# Autodesk Inventor assembly: belt_liner-2-1
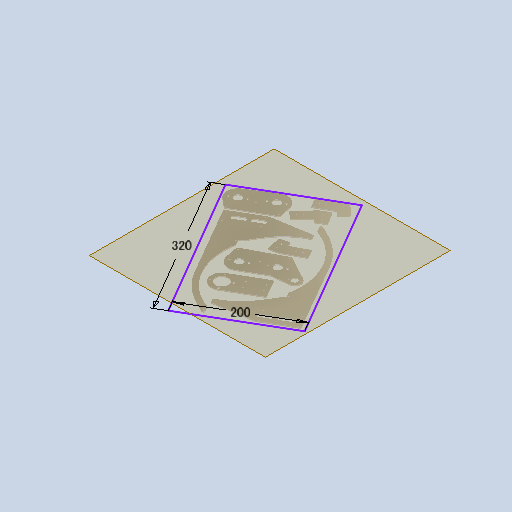
[picture p0: Inventor's stored thumbnail of the model, 512x512]
Saved by Autodesk Inventor 2025.2 (Build 292293000, 293)
## iProperties
Created: 2025-01-15
Part Number: belt_liner-2-1
Document SubType Name: Assembly
Designer: haruy
Author: haruy
## Documents named in this file (7)
- C:\Users\haruy\Documents\ロボコン\NHK2025\cad\cnc\belt_liner-2-1.iam
- C:\Users\haruy\Documents\ロボコン\NHK2025\cad\nagahisa\belt_liner\belt_liner_v2_Plate_6.ipt
- C:\Users\haruy\Documents\ロボコン\NHK2025\cad\nagahisa\belt_liner\belt_liner_v2_Plate_15.ipt
- C:\Users\haruy\Documents\ロボコン\NHK2025\cad\nagahisa\belt_liner\belt_liner_v2_Plate_17.ipt
- C:\Users\haruy\Documents\ロボコン\NHK2025\cad\nagahisa\belt_liner\belt_liner_v2_Plate_16.ipt
- C:\Users\haruy\Documents\ロボコン\NHK2025\cad\nagahisa\dribl\dribl-v1-Plate-10.ipt
- C:\Users\haruy\Documents\ロボコン\NHK2025\cad\nagahisa\dribl\dribl-v1-Plate-11.ipt
## Components (8 placed, 6 different names)
1. belt_liner_v2_Plate_6:1 — フラッシュ:1, 角度:1, 角度:2, 角度:3
2. belt_liner_v2_Plate_6:2 — フラッシュ:2, 角度:1, メイト:1
3. belt_liner_v2_Plate_15:1 — フラッシュ:3, 角度:2
4. belt_liner_v2_Plate_17:1 — フラッシュ:4, メイト:2
5. belt_liner_v2_Plate_16:1 — フラッシュ:5, メイト:1
6. dribl-v1-Plate-10:1 — フラッシュ:6, メイト:2
7. dribl-v1-Plate-10:2 — フラッシュ:7, 角度:3, メイト:3
8. dribl-v1-Plate-11:1 — フラッシュ:8, メイト:3
## Relationships (14: Flush 8, Angle 3, Mate 3)
- フラッシュ:1 [Flush]: belt_liner_v2_Plate_6:1
- フラッシュ:2 [Flush]: belt_liner_v2_Plate_6:2
- 角度:1 [Angle] (180 deg): belt_liner_v2_Plate_6:1 ↔ belt_liner_v2_Plate_6:2
- フラッシュ:3 [Flush]: belt_liner_v2_Plate_15:1
- 角度:2 [Angle] (0 deg): belt_liner_v2_Plate_6:1 ↔ belt_liner_v2_Plate_15:1
- フラッシュ:4 [Flush]: belt_liner_v2_Plate_17:1
- フラッシュ:5 [Flush]: belt_liner_v2_Plate_16:1
- メイト:1 [Mate] (5 mm): belt_liner_v2_Plate_6:2 ↔ belt_liner_v2_Plate_16:1
- フラッシュ:6 [Flush]: dribl-v1-Plate-10:1
- メイト:2 [Mate] (5 mm): belt_liner_v2_Plate_17:1 ↔ dribl-v1-Plate-10:1
- フラッシュ:7 [Flush]: dribl-v1-Plate-10:2
- 角度:3 [Angle] (0 deg): belt_liner_v2_Plate_6:1 ↔ dribl-v1-Plate-10:2
- フラッシュ:8 [Flush]: dribl-v1-Plate-11:1
- メイト:3 [Mate] (5 mm): dribl-v1-Plate-10:2 ↔ dribl-v1-Plate-11:1
